# Autodesk Inventor assembly: Link2
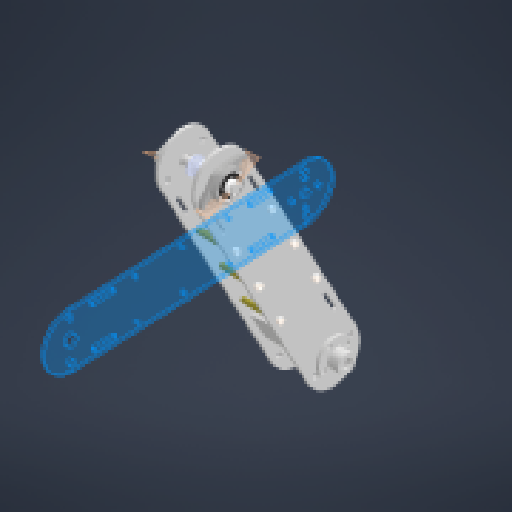
[picture p0: Inventor's stored thumbnail of the model, 512x512]
Saved by Autodesk Inventor 2023 (Build 270158000, 158)
## iProperties
Created: 2023-09-09
Part Number: Link2
Document SubType Name: Assembly
Designer: philo
Author: philo
## Documents named in this file (10)
- C:\Users\philo\OneDrive\Desktop\HK1-2024\TT ROBOT\02_3D_design_new\Link2.iam
- C:\Users\philo\OneDrive\Desktop\HK1-2024\TT ROBOT\02_3D_design_new\Link2Base.ipt
- C:\Users\philo\OneDrive\Desktop\HK1-2024\TT ROBOT\02_3D_design_new\goidoObi.ipt
- C:\Users\philo\OneDrive\Desktop\HK1-2024\TT ROBOT\02_3D_design_new\truc8mm.ipt
- C:\Users\philo\OneDrive\Desktop\HK1-2024\TT ROBOT\02_3D_design_new\GT2 Pulley 20 Tooth (ID6mm).ipt
- C:\Users\philo\OneDrive\Desktop\HK1-2024\TT ROBOT\02_3D_design_new\trudong3mm.ipt
- C:\Users\philo\OneDrive\Desktop\HK1-2024\TT ROBOT\02_3D_design_new\M3 x 5mm.ipt
- C:\Users\philo\OneDrive\Desktop\HK1-2024\TT ROBOT\02_3D_design_new\codinhtruc.ipt
- C:\Users\philo\OneDrive\Desktop\HK1-2024\TT ROBOT\02_3D_design_new\60pitch pulley GT2 6mm ASSEMBLY.iam
- C:\Users\philo\OneDrive\Desktop\HK1-2024\TT ROBOT\02_3D_design_new\Dongco.iam
## Components (28 placed, 9 different names)
1. GT2 Pulley 20 Tooth (ID6mm):1 — Mate:80, Mate:81
2. Dongco:1 [sub-assembly] — Mate:78, Angle:3, Mate:79, Mate:80
3. 60pitch pulley GT2 6mm ASSEMBLY:1 [sub-assembly] — Mate:76, Mate:77
4. Link2Base:2 — Mate:54, Mate:55, Mate:56, Mate:57, Mate:58, Mate:59, Mate:60, Mate:61, Mate:62, Mate:63, Mate:64, Mate:65, Mate:71, Mate:72, Mate:73, Mate:74, Mate:75, Angle:2, Mate:78, Mate:79, Mate:81
5. Link2Base:3 — Mate:68, Mate:69, Mate:70, Mate:77, Angle:3
6. goidoObi:2
7. truc8mm:1 — Mate:76
8. trudong3mm:1 — Mate:66
9. trudong3mm:2
10. trudong3mm:3
11. trudong3mm:4
12. trudong3mm:5
13. trudong3mm:6 — Mate:67
14. M3 x 5mm:1
15. M3 x 5mm:2
16. M3 x 5mm:3
17. M3 x 5mm:4 — Mate:66
18. M3 x 5mm:5
19. M3 x 5mm:6
20. M3 x 5mm:7 — Mate:54, Mate:55
21. M3 x 5mm:8 — Mate:62, Mate:63, Mate:67
22. M3 x 5mm:9 — Mate:64, Mate:65
23. M3 x 5mm:10 — Mate:56, Mate:57
24. M3 x 5mm:11 — Mate:58, Mate:59
25. M3 x 5mm:12 — Mate:60, Mate:61
26. goidoObi:3 — Mate:74, Mate:75, Angle:2
27. codinhtruc:1 — Mate:68, Mate:69, Mate:70
28. codinhtruc:2 — Mate:71, Mate:72, Mate:73
## Relationships (59: Mate 55, Angle 3, Flush 1)
- [Mate] (30 mm): Link2Base:2 ↔ Link2Base:3
- [Mate]: Link2Base:3 ↔ goidoObi:2
- [Mate]: Link2Base:3 ↔ goidoObi:2
- [Angle] (90 deg): Link2Base:3 ↔ goidoObi:2
- [Flush] (-35 mm): goidoObi:2 ↔ truc8mm:1
- [Mate]: Link2Base:2 ↔ trudong3mm:1
- [Mate]: Link2Base:3 ↔ trudong3mm:1
- [Mate]: Link2Base:3 ↔ trudong3mm:3
- [Mate]: Link2Base:3 ↔ trudong3mm:4
- [Mate]: Link2Base:3 ↔ trudong3mm:2
- [Mate]: Link2Base:3 ↔ trudong3mm:5
- [Mate]: Link2Base:3 ↔ trudong3mm:5
- [Mate]: Link2Base:3 ↔ trudong3mm:2
- [Mate]: Link2Base:3 ↔ trudong3mm:4
- [Mate]: Link2Base:3 ↔ trudong3mm:3
- [Mate]: Link2Base:2 ↔ trudong3mm:6
- [Mate]: Link2Base:3 ↔ M3 x 5mm:1
- [Mate]: Link2Base:3 ↔ M3 x 5mm:1
- [Mate]: Link2Base:3 ↔ M3 x 5mm:2
- [Mate]: Link2Base:3 ↔ M3 x 5mm:3
- [Mate]: Link2Base:3 ↔ M3 x 5mm:4
- [Mate]: Link2Base:3 ↔ M3 x 5mm:5
- [Mate]: Link2Base:3 ↔ M3 x 5mm:4
- [Mate]: Link2Base:3 ↔ M3 x 5mm:3
- [Mate]: Link2Base:3 ↔ M3 x 5mm:2
- [Mate]: Link2Base:3 ↔ M3 x 5mm:5
- [Mate]: Link2Base:3 ↔ M3 x 5mm:6
- [Mate]: Link2Base:3 ↔ M3 x 5mm:6
- [Mate]: goidoObi:2 ↔ truc8mm:1
- Mate:54: Link2Base:2 ↔ M3 x 5mm:7
- Mate:55: Link2Base:2 ↔ M3 x 5mm:7
- Mate:56: Link2Base:2 ↔ M3 x 5mm:10
- Mate:57: Link2Base:2 ↔ M3 x 5mm:10
- Mate:58: Link2Base:2 ↔ M3 x 5mm:11
- Mate:59: Link2Base:2 ↔ M3 x 5mm:11
- Mate:60: Link2Base:2 ↔ M3 x 5mm:12
- Mate:61: Link2Base:2 ↔ M3 x 5mm:12
- Mate:62: Link2Base:2 ↔ M3 x 5mm:8
- Mate:63: Link2Base:2 ↔ M3 x 5mm:8
- Mate:64: Link2Base:2 ↔ M3 x 5mm:9
- Mate:65: Link2Base:2 ↔ M3 x 5mm:9
- Mate:66: trudong3mm:1 ↔ M3 x 5mm:4
- Mate:67: trudong3mm:6 ↔ M3 x 5mm:8
- Mate:68: Link2Base:3 ↔ codinhtruc:1
- Mate:69: Link2Base:3 ↔ codinhtruc:1
- Mate:70: Link2Base:3 ↔ codinhtruc:1
- Mate:71: Link2Base:2 ↔ codinhtruc:2
- Mate:72: Link2Base:2 ↔ codinhtruc:2
- Mate:73: Link2Base:2 ↔ codinhtruc:2
- Mate:74: Link2Base:2 ↔ goidoObi:3
- Mate:75: Link2Base:2 ↔ goidoObi:3
- Angle:2 (0 deg): Link2Base:2 ↔ goidoObi:3
- Mate:76: 60pitch pulley GT2 6mm ASSEMBLY:1 ↔ truc8mm:1
- Mate:77 (10 mm): 60pitch pulley GT2 6mm ASSEMBLY:1 ↔ Link2Base:3
- Mate:78: Dongco:1 ↔ Link2Base:2
- Angle:3 (0 deg): Dongco:1 ↔ Link2Base:3
- Mate:79: Dongco:1 ↔ Link2Base:2
- Mate:80: GT2 Pulley 20 Tooth (ID6mm):1 ↔ Dongco:1
- Mate:81 (2 mm): GT2 Pulley 20 Tooth (ID6mm):1 ↔ Link2Base:2
